# Autodesk Inventor assembly: bracket_assy
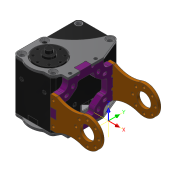
[picture p0: Inventor's stored thumbnail of the model, 180x180]
Saved by Autodesk Inventor 2019.4 (Build 234330000, 330)
## iProperties
Created: 2018-04-26
Part Number: bracket_assy
Material: 一般
Document SubType Name: Assembly
Designer: cmflab
Mass: 88.3973 g
Surface Area: 206.931 cm^2
Volume: 50.433 cm^3
Density: 1.75277 g/cm^3
Author: cmflab
## Documents named in this file (6)
- C:\Workspace\HaptHexa\Hardware\Inventor\Coxa\_Coxa.iam
- C:\Workspace\HaptHexa\Hardware\Inventor\Coxa\tap_block.ipt
- C:\Workspace\HaptHexa\Hardware\Inventor\Coxa\tab_yaw_top.ipt
- C:\Workspace\HaptHexa\Hardware\Inventor\Coxa\tab_pitch_out.ipt
- C:\Workspace\HaptHexa\Hardware\Inventor\Coxa\tab_pitch_out_mir.ipt
- C:\Workspace\HaptHexa\Hardware\Inventor\X430\x-430_idle.iam
## Components (6 placed, 5 different names)
1. tap_block:1 — メイト:1, メイト:2, メイト:3, メイト:4, メイト:5, メイト:6, メイト:7, メイト:8, メイト:9, メイト:15, メイト:16, メイト:17, フラッシュ:1, フラッシュ:2
2. tab_yaw_top:1 — メイト:1, メイト:2, メイト:6
3. tab_yaw_top:2 — メイト:4, メイト:5, メイト:3, メイト:13
4. tab_pitch_out:1 — メイト:7, メイト:8, メイト:9, メイト:18, メイト:19, メイト:20
5. tab_pitch_out_mir:1 — メイト:15, メイト:16, メイト:17
6. x-430_idle:1 [sub-assembly] — メイト:18, メイト:19, メイト:20
## Relationships (18: Mate 16, Flush 2)
- メイト:1 [Mate]: tap_block:1 ↔ tab_yaw_top:1
- メイト:2 [Mate]: tap_block:1 ↔ tab_yaw_top:1
- メイト:3 [Mate]: tap_block:1 ↔ tab_yaw_top:2
- メイト:4 [Mate]: tap_block:1 ↔ tab_yaw_top:2
- メイト:5 [Mate]: tap_block:1 ↔ tab_yaw_top:2
- メイト:6 [Mate]: tap_block:1 ↔ tab_yaw_top:1
- メイト:7 [Mate]: tap_block:1 ↔ tab_pitch_out:1
- メイト:8 [Mate]: tap_block:1 ↔ tab_pitch_out:1
- メイト:9 [Mate]: tap_block:1 ↔ tab_pitch_out:1
- メイト:13 [Mate]: tab_yaw_top:2
- メイト:15 [Mate]: tap_block:1 ↔ tab_pitch_out_mir:1
- メイト:16 [Mate]: tap_block:1 ↔ tab_pitch_out_mir:1
- メイト:17 [Mate]: tap_block:1 ↔ tab_pitch_out_mir:1
- フラッシュ:1 [Flush] (6 mm): tap_block:1
- フラッシュ:2 [Flush]: tap_block:1
- メイト:18 [Mate]: tab_pitch_out:1 ↔ x-430_idle:1
- メイト:19 [Mate]: tab_pitch_out:1 ↔ x-430_idle:1
- メイト:20 [Mate]: tab_pitch_out:1 ↔ x-430_idle:1
## Named parameters: sa_0 = 50, sa_1 = 2e-13, sa_2 = 500, sa_3 = 0
note: some values were not read from the file. Shown as the stored number, unit unknown: "sa_0", "sa_1", "sa_2", "sa_3".
